# Autodesk Inventor assembly: Pneumatics Assembly
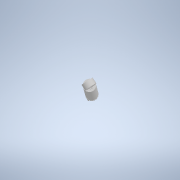
[picture p0: Inventor's stored thumbnail of the model, 180x180]
Saved by Autodesk Inventor 2020 (Build 240168000, 168)
## iProperties
Created: 2021-01-30
Part Number: Pneumatics Assembly
Document SubType Name: Assembly
Designer: magda
Author: magda
## Documents named in this file (5)
- C:\Users\magda\OneDrive\Documents\Inventor\T3\Ramp Intake\Pneumatics Assembly.iam
- C:\Users\magda\OneDrive\Documents\Inventor\T3\Ramp Intake\Exterior Pneumatics cell.ipt
- C:\Users\magda\OneDrive\Documents\Inventor\T3\Ramp Intake\Interior Pneumatics Cell.ipt
- C:\Users\magda\OneDrive\Documents\Inventor\T3\Ramp Intake\Load Notch Insert.ipt
- C:\Users\magda\OneDrive\Documents\Inventor\T3\Ramp Intake\Bottom Pneumatics notch.ipt
## Components (4 placed, 4 different names)
1. Exterior Pneumatics cell:1 — Mate:1, Mate:4, Mate:5
2. Interior Pneumatics Cell:1 — Mate:1, Mate:2, Mate:3
3. Load Notch Insert:1 — Mate:2, Mate:3
4. Bottom Pneumatics notch:1 — Mate:4, Mate:5
## Relationships (5: Mate 5)
- Mate:1: Exterior Pneumatics cell:1 ↔ Interior Pneumatics Cell:1
- Mate:2: Interior Pneumatics Cell:1 ↔ Load Notch Insert:1
- Mate:3: Interior Pneumatics Cell:1 ↔ Load Notch Insert:1
- Mate:4: Exterior Pneumatics cell:1 ↔ Bottom Pneumatics notch:1
- Mate:5: Exterior Pneumatics cell:1 ↔ Bottom Pneumatics notch:1
